# Autodesk Inventor assembly: Ensamblaje prueba
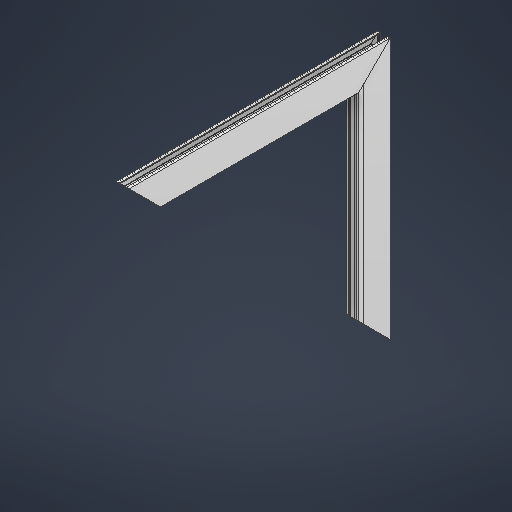
[picture p0: Inventor's stored thumbnail of the model, 512x512]
Saved by Autodesk Inventor 2025 (Build 290162000, 162)
## iProperties
Created: 2026-02-05
Part Number: Ensamblaje prueba
Document SubType Name: Assembly
Designer: ROLANDO
Mass: 807.458 g
Surface Area: 3974.28 cm^2
Volume: 300.087 cm^3
Density: 2.69075 g/cm^3
Author: ROLANDO
## Documents named in this file (4)
- C:\Users\rolan\OneDrive\Documentos\Inventor\Projects\CARPINTERIA ALUMINIO\PUERTAS Y VENTANAS\Ensamblaje prueba.iam
- C:\Users\rolan\OneDrive\Documentos\Inventor\Projects\CARPINTERIA ALUMINIO\PUERTAS Y VENTANAS\ESCUADRAS\ESCUADRA UNIÓN 45 DISEÑO NUEVO.ipt
- C:\Users\rolan\OneDrive\Documentos\Inventor\Projects\CARPINTERIA ALUMINIO\PUERTAS Y VENTANAS\ENSAMBLE PRUEBA SP40-04A TRAVESAÑO CENTRAL.ipt
- C:\Users\rolan\OneDrive\Documentos\Inventor\Projects\CARPINTERIA ALUMINIO\PUERTAS Y VENTANAS\TORNILLO DE PRUEBA.ipt
## Components (5 placed, 3 different names)
1. ESCUADRA UNIÓN 45 DISEÑO NUEVO:1 — Nivelación:1, Coincidencia:1, Nivelación:2, Coincidencia:4
2. ENSAMBLE PRUEBA SP40-04A TRAVESAÑO CENTRAL:1 — Nivelación:1, Coincidencia:1, Coincidencia:2, Coincidencia:3, Insertar:4
3. ENSAMBLE PRUEBA SP40-04A TRAVESAÑO CENTRAL:2 — Nivelación:2, Coincidencia:2, Coincidencia:3, Coincidencia:4, Insertar:5
4. TORNILLO DE PRUEBA:1 — Insertar:4
5. TORNILLO DE PRUEBA:2 — Insertar:5
## Relationships (8: Mate 4, Flush 2, Insert 2)
- Nivelación:1 [Flush]: ESCUADRA UNIÓN 45 DISEÑO NUEVO:1 ↔ ENSAMBLE PRUEBA SP40-04A TRAVESAÑO CENTRAL:1
- Coincidencia:1 [Mate] (0.6 mm): ESCUADRA UNIÓN 45 DISEÑO NUEVO:1 ↔ ENSAMBLE PRUEBA SP40-04A TRAVESAÑO CENTRAL:1
- Nivelación:2 [Flush]: ESCUADRA UNIÓN 45 DISEÑO NUEVO:1 ↔ ENSAMBLE PRUEBA SP40-04A TRAVESAÑO CENTRAL:2
- Coincidencia:2 [Mate]: ENSAMBLE PRUEBA SP40-04A TRAVESAÑO CENTRAL:1 ↔ ENSAMBLE PRUEBA SP40-04A TRAVESAÑO CENTRAL:2
- Coincidencia:3 [Mate]: ENSAMBLE PRUEBA SP40-04A TRAVESAÑO CENTRAL:1 ↔ ENSAMBLE PRUEBA SP40-04A TRAVESAÑO CENTRAL:2
- Coincidencia:4 [Mate] (0.6 mm): ESCUADRA UNIÓN 45 DISEÑO NUEVO:1 ↔ ENSAMBLE PRUEBA SP40-04A TRAVESAÑO CENTRAL:2
- Insertar:4: ENSAMBLE PRUEBA SP40-04A TRAVESAÑO CENTRAL:1 ↔ TORNILLO DE PRUEBA:1
- Insertar:5: ENSAMBLE PRUEBA SP40-04A TRAVESAÑO CENTRAL:2 ↔ TORNILLO DE PRUEBA:2
